# Autodesk Inventor assembly: Nose cam assy
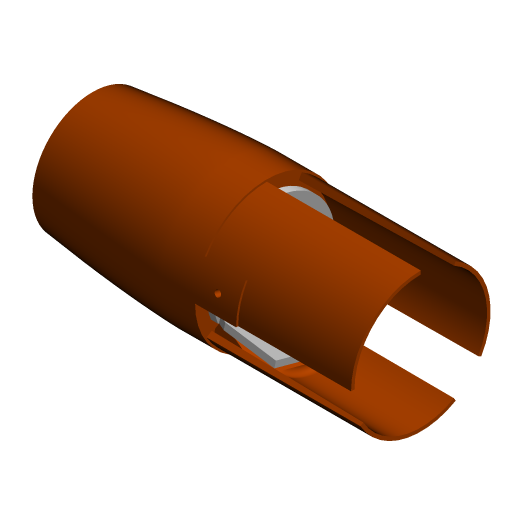
[picture p0: Inventor's stored thumbnail of the model, 512x512]
Saved by Autodesk Inventor 2024 (Build 280153000, 153)
## iProperties
Part Number: Nose cam assy
Document SubType Name: Assembly
Designer: Jamie
Author: Jamie
## Documents named in this file (3)
- C:\Users\Jamie\Documents\Uni\DARE\Scrambler-2-CAD\Autodesk\Nose cam assy.iam
- C:\Users\Jamie\Documents\Uni\DARE\Scrambler-2-CAD\Autodesk\Nose cam retention.ipt
- C:\Users\Jamie\Documents\Uni\DARE\Scrambler-2-CAD\Autodesk\Nosecone base with cam.ipt
## Components (2 placed, 2 different names)
1. Nose cam retention:1 — Mate:1, Mate:2, Angle:1
2. Nosecone base with cam:1 — Mate:1, Mate:2, Angle:1
## Relationships (3: Mate 2, Angle 1)
- Mate:1: Nose cam retention:1 ↔ Nosecone base with cam:1
- Mate:2: Nose cam retention:1 ↔ Nosecone base with cam:1
- Angle:1 (180 deg): Nose cam retention:1 ↔ Nosecone base with cam:1
